# Autodesk Inventor assembly: CL3-100
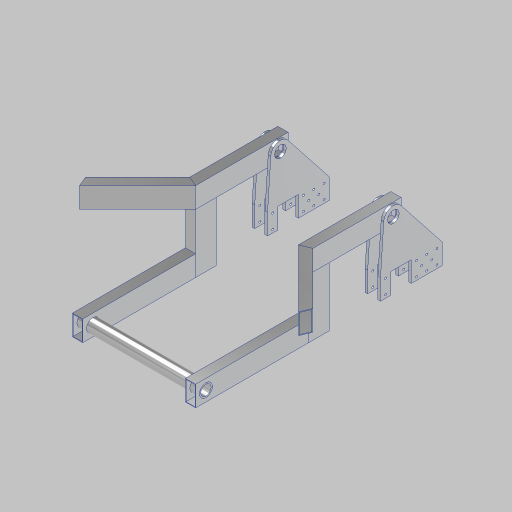
[picture p0: Inventor's stored thumbnail of the model, 512x512]
Saved by Autodesk Inventor 2023.5 (Build 275446000, 446)
## iProperties
Created: 2025-01-28
Part Number: CL3-100
Document SubType Name: Assembly
Designer: slick
Mass: 5241.21 g
Surface Area: 12801.1 cm^2
Volume: 1941.19 cm^3
Density: 2.7 g/cm^3
Author: slick
## Documents named in this file (8)
- C:\Users\slick\OneDrive\Desktop\2025-ReefScape---CAD\Climber\CL3\CL3-100.iam
- C:\Users\slick\OneDrive\Desktop\2025-ReefScape---CAD\Climber\CL3\CL3-001.ipt
- C:\Users\slick\OneDrive\Desktop\2025-ReefScape---CAD\Climber\CL3\CL3-002.ipt
- C:\Users\slick\OneDrive\Desktop\2025-ReefScape---CAD\Climber\CL3\CL3-003.ipt
- C:\Users\slick\OneDrive\Desktop\2025-ReefScape---CAD\Climber\CL3\CL3-004.ipt
- C:\Users\slick\OneDrive\Desktop\2025-ReefScape---CAD\Climber\CL3\CL3-006.ipt
- C:\Users\slick\OneDrive\Desktop\2025-ReefScape---CAD\Field Items\Full Field\FE-2025\GE-25201.iam
- C:\Users\slick\OneDrive\Desktop\2025-ReefScape---CAD\Climber\CL3\CL3-007.ipt
## Components (14 placed, 7 different names)
1. CL3-001:1 — Mate:9, Flush:5, Mate:10, Mate:11, Mate:15, Mate:16, Symmetry:1, Mate:22, Flush:14, Angle:1, Mate:24, Flush:24, Mate:25, Mate:28
2. CL3-002:1 — Mate:24, Flush:24, Mate:25
3. CL3-003:1 — Mate:19, Flush:28, Flush:29, Mate:30, Flush:30
4. CL3-001:2 — Mate:9, Flush:5, Mate:13, Mate:14, Mate:17, Symmetry:1, Mate:23, Flush:13, Mate:26, Flush:25, Mate:27
5. CL3-002:2 — Mate:26, Flush:25, Mate:27
6. CL3-003:2 — Mate:29, Flush:26, Flush:27, Flush:28
7. CL3-004:1 — Flush:7, Mate:12, Mate:13, Flush:9, Mate:17
8. CL3-004:2 — Flush:7, Mate:10, Mate:15, Flush:8, Flush:23
9. CL3-004:3 — Mate:11, Mate:16, Flush:8, Angle:1
10. CL3-004:4 — Mate:12, Mate:14, Flush:9, Flush:23
11. CL3-006:1 — Mate:19, Tangent:1, Mate:21, Flush:30
12. GE-25201:1 [sub-assembly] — Mate:20, Tangent:1, Mate:21
13. CL3-007:1 — Mate:22, Flush:14, Flush:15, Mate:28, Mate:29, Flush:26, Flush:27
14. CL3-007:2 — Mate:23, Flush:13, Flush:15, Flush:29, Mate:30
## Relationships (39: Mate 21, Flush 15, Symmetry 1, Tangent 1, Angle 1)
- Mate:9 (254 mm): CL3-001:1 ↔ CL3-001:2
- Flush:5: CL3-001:1 ↔ CL3-001:2
- Flush:7: CL3-004:1 ↔ CL3-004:2
- Mate:10: CL3-001:1 ↔ CL3-004:2
- Mate:11: CL3-001:1 ↔ CL3-004:3
- Mate:12: CL3-004:1 ↔ CL3-004:4
- Mate:13: CL3-001:2 ↔ CL3-004:1
- Mate:14: CL3-001:2 ↔ CL3-004:4
- Mate:15: CL3-001:1 ↔ CL3-004:2
- Mate:16: CL3-001:1 ↔ CL3-004:3
- Flush:8: CL3-004:2 ↔ CL3-004:3
- Flush:9: CL3-004:1 ↔ CL3-004:4
- Mate:17: CL3-001:2 ↔ CL3-004:1
- Mate:19: CL3-003:1 ↔ CL3-006:1
- Symmetry:1: CL3-001:1 ↔ CL3-001:2
- Mate:20: GE-25201:1
- Tangent:1: CL3-006:1 ↔ GE-25201:1
- Mate:21 (-76.2 mm): CL3-006:1 ↔ GE-25201:1
- Mate:22: CL3-001:1 ↔ CL3-007:1
- Mate:23: CL3-001:2 ↔ CL3-007:2
- Flush:13: CL3-001:2 ↔ CL3-007:2
- Flush:14: CL3-001:1 ↔ CL3-007:1
- Flush:15: CL3-007:1 ↔ CL3-007:2
- Flush:23: CL3-004:2 ↔ CL3-004:4
- Angle:1 (90 deg): CL3-001:1 ↔ CL3-004:3
- Mate:24: CL3-001:1 ↔ CL3-002:1
- Flush:24: CL3-001:1 ↔ CL3-002:1
- Mate:25: CL3-001:1 ↔ CL3-002:1
- Mate:26: CL3-001:2 ↔ CL3-002:2
- Flush:25: CL3-001:2 ↔ CL3-002:2
- Mate:27: CL3-001:2 ↔ CL3-002:2
- Mate:28: CL3-001:1 ↔ CL3-007:1
- Mate:29: CL3-003:2 ↔ CL3-007:1
- Flush:26: CL3-003:2 ↔ CL3-007:1
- Flush:27: CL3-003:2 ↔ CL3-007:1
- Flush:28: CL3-003:1 ↔ CL3-003:2
- Flush:29: CL3-003:1 ↔ CL3-007:2
- Mate:30: CL3-003:1 ↔ CL3-007:2
- Flush:30: CL3-003:1 ↔ CL3-006:1
